# Autodesk Inventor assembly: 全体v1
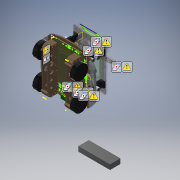
[picture p0: Inventor's stored thumbnail of the model, 180x180]
Saved by Autodesk Inventor 2018.3 (Build 223284000, 284)
## iProperties
Created: 2018-11-27
Part Number: 全体v1
Material: 一般
Document SubType Name: Assembly
Designer: shun2
Author: shun2
## Documents named in this file (27)
- C:\Users\shun2\OneDrive\おそらく最新版(2018.7.31)\全体v1.iam
- C:\Users\shun2\OneDrive\おそらく最新版(2018.7.31)\ギアボックス\ギアボックスv2.iam
- C:\Users\shun2\OneDrive\おそらく最新版(2018.7.31)\1枚目\一枚目.ipt
- C:\Users\shun2\OneDrive\おそらく最新版(2018.7.31)\基板保護2018.8.7.ipt
- C:\Users\shun2\OneDrive\おそらく最新版(2018.7.31)\2枚目\2枚目.ipt
- C:\Users\shun2\OneDrive\おそらく最新版(2018.7.31)\3枚目\3枚目v4.ipt
- C:\Users\shun2\OneDrive\おそらく最新版(2018.7.31)\ping-module.iam
- C:\Users\shun2\OneDrive\おそらく最新版(2018.7.31)\pingmodule-y.iam
- C:\Users\shun2\OneDrive\おそらく最新版(2018.7.31)\Color.ipt
- C:\Users\shun2\OneDrive\おそらく最新版(2018.7.31)\モタドラ.ipt
- C:\Users\shun2\OneDrive\おそらく最新版(2018.7.31)\メイン基板.ipt
- C:\Users\shun2\OneDrive\おそらく最新版(2018.7.31)\Aquila-2018-Under.ipt
- C:\Users\shun2\OneDrive\おそらく最新版(2018.7.31)\LiFePo.ipt
- C:\Users\shun2\OneDrive\おそらく最新版(2018.7.31)\LiFeGuard.ipt
- C:\Users\shun2\OneDrive\おそらく最新版(2018.7.31)\Ping-front.ipt
- C:\Users\shun2\OneDrive\おそらく最新版(2018.7.31)\Tire.ipt
- C:\Users\shun2\OneDrive\おそらく最新版(2018.7.31)\レスキューキット投下機構\RescueKit-Pipev3.ipt
- C:\Users\shun2\OneDrive\おそらく最新版(2018.7.31)\レスキューキット投下機構\RescueKit-Slidev2.ipt
- C:\Users\shun2\OneDrive\おそらく最新版(2018.7.31)\レスキューキット投下機構\28BYJ-48.ipt
- C:\Users\shun2\OneDrive\おそらく最新版(2018.7.31)\レスキューキット投下機構\RescueKit-Gear-18.ipt
- C:\Users\shun2\OneDrive\おそらく最新版(2018.7.31)\UI固定具.ipt
- C:\Users\shun2\OneDrive\おそらく最新版(2018.7.31)\M024-ILI9328 data.ipt
- C:\Users\shun2\OneDrive\おそらく最新版(2018.7.31)\GyroMountv2.ipt
- C:\Users\shun2\OneDrive\おそらく最新版(2018.7.31)\OpenMVMount-Tate-Shortv2.ipt
- C:\Users\shun2\OneDrive\おそらく最新版(2018.7.31)\OpenMVMount-Tatev2.ipt
- C:\Users\shun2\OneDrive\おそらく最新版(2018.7.31)\ping.ipt
- C:\Users\shun2\OneDrive\おそらく最新版(2018.7.31)\ガイド\ガイド横上.ipt
## Components (34 placed, 26 different names)
1. 一枚目:1 — メイト:1, メイト:2, フラッシュ:1, フラッシュ:2, フラッシュ:3, フラッシュ:4, メイト:3, メイト:4, メイト:5, メイト:44, メイト:45, メイト:46, メイト:47, メイト:48, メイト:49, メイト:53, メイト:54, メイト:55, メイト:95, メイト:151
2. 2枚目:1 — メイト:6, メイト:7, メイト:8, メイト:41, メイト:42, メイト:94, メイト:108, メイト:109, メイト:110, メイト:127, メイト:157, メイト:158, メイト:179, メイト:180, メイト:181, メイト:187, メイト:188, メイト:189, メイト:190, メイト:191, メイト:192
3. 3枚目v4:1 — メイト:41, メイト:42, メイト:50, メイト:94, メイト:127, メイト:132, メイト:133, メイト:134, メイト:135, メイト:136, メイト:137, メイト:138, メイト:139, メイト:140, メイト:141, メイト:142, メイト:143, メイト:144, メイト:145, メイト:146, メイト:159, メイト:160, メイト:161, メイト:162, メイト:163, メイト:164, メイト:165, メイト:166, メイト:177, メイト:178, メイト:182, メイト:183
4. 基板保護2018.8.7:1 — メイト:3, メイト:4, メイト:5, メイト:6, メイト:7, メイト:8
5. LiFePo:1
6. LiFeGuard:2 — メイト:108, メイト:109, メイト:110
7. RescueKit-Slidev2:1 — メイト:157
8. 28BYJ-48:1 — メイト:152, メイト:153, メイト:158
9. RescueKit-Gear-18:1 — メイト:152, メイト:153
10. RescueKit-Pipev3:1 — メイト:159, メイト:160, メイト:161
11. UI固定具:1 — メイト:164, メイト:165, メイト:166, メイト:168, メイト:169, メイト:170, メイト:171, メイト:172, メイト:173
12. M024-ILI9328 data:1 — メイト:168, メイト:169, メイト:170
13. GyroMountv2:1 — メイト:171, メイト:172, メイト:173
14. OpenMVMount-Tatev2:1 — メイト:177, メイト:178
15. Ping-front:1 — メイト:179, メイト:180, メイト:181, メイト:184, メイト:185, メイト:186
16. OpenMVMount-Tate-Shortv2:1 — メイト:182, メイト:183
17. ping:1 — メイト:184, メイト:185, メイト:186
18. ガイド横上:1 — メイト:187, メイト:188, メイト:189
19. ガイド横上:2 — メイト:190, メイト:191, メイト:192
20. ping-module:1 [sub-assembly] — メイト:132, メイト:133, メイト:134
21. ping-module:2 [sub-assembly] — メイト:141, メイト:142, メイト:143
22. ping-module:3 [sub-assembly] — メイト:138, メイト:139, メイト:140
23. ping-module:4 [sub-assembly] — メイト:135, メイト:136, メイト:137
24. pingmodule-y:1 [sub-assembly] — メイト:144, メイト:145, メイト:146
25. Color:1 — メイト:44, メイト:45, メイト:46
26. モタドラ:1 — メイト:47, メイト:48, メイト:49
27. メイン基板:1 — メイト:50, メイト:162, メイト:163
28. Aquila-2018-Under:2 — メイト:53, メイト:54, メイト:55
29. Tire:1 — メイト:86, メイト:87
30. Tire:2 — メイト:88, メイト:89
31. Tire:3 — メイト:92, メイト:93
32. Tire:4 — メイト:90, メイト:91
33. ギアボックスv2:2 [sub-assembly] — メイト:2, フラッシュ:1, フラッシュ:4, メイト:86, メイト:87, メイト:88, メイト:89
34. ギアボックスv2:1 [sub-assembly] — メイト:1, フラッシュ:2, フラッシュ:3, メイト:90, メイト:91, メイト:92, メイト:93, メイト:96
## Relationships (89: Mate 85, Flush 4)
- メイト:1 [Mate] (3 mm): 一枚目:1 ↔ ギアボックスv2:1
- メイト:2 [Mate] (3 mm): 一枚目:1 ↔ ギアボックスv2:2
- フラッシュ:1 [Flush]: 一枚目:1 ↔ ギアボックスv2:2
- フラッシュ:2 [Flush]: 一枚目:1 ↔ ギアボックスv2:1
- フラッシュ:3 [Flush] (2 mm): 一枚目:1 ↔ ギアボックスv2:1
- フラッシュ:4 [Flush] (2 mm): 一枚目:1 ↔ ギアボックスv2:2
- メイト:3 [Mate] (0.2 mm): 一枚目:1 ↔ 基板保護2018.8.7:1
- メイト:4 [Mate]: 一枚目:1 ↔ 基板保護2018.8.7:1
- メイト:5 [Mate]: 一枚目:1 ↔ 基板保護2018.8.7:1
- メイト:6 [Mate] (3 mm): 2枚目:1 ↔ 基板保護2018.8.7:1
- メイト:7 [Mate]: 2枚目:1 ↔ 基板保護2018.8.7:1
- メイト:8 [Mate]: 2枚目:1 ↔ 基板保護2018.8.7:1
- メイト:41 [Mate] (80 mm): 2枚目:1 ↔ 3枚目v4:1
- メイト:42 [Mate]: 2枚目:1 ↔ 3枚目v4:1
- メイト:44 [Mate] (40 mm): 一枚目:1 ↔ Color:1
- メイト:45 [Mate]: 一枚目:1 ↔ Color:1
- メイト:46 [Mate]: 一枚目:1 ↔ Color:1
- メイト:47 [Mate] (8 mm): 一枚目:1 ↔ モタドラ:1
- メイト:48 [Mate]: 一枚目:1 ↔ モタドラ:1
- メイト:49 [Mate]: 一枚目:1 ↔ モタドラ:1
- メイト:50 [Mate] (8 mm): 3枚目v4:1 ↔ メイン基板:1
- メイト:53 [Mate] (3 mm): 一枚目:1 ↔ Aquila-2018-Under:2
- メイト:54 [Mate]: 一枚目:1 ↔ Aquila-2018-Under:2
- メイト:55 [Mate]: 一枚目:1 ↔ Aquila-2018-Under:2
- メイト:86 [Mate] (8 mm): Tire:1 ↔ ギアボックスv2:2
- メイト:87 [Mate]: Tire:1 ↔ ギアボックスv2:2
- メイト:88 [Mate] (8 mm): Tire:2 ↔ ギアボックスv2:2
- メイト:89 [Mate]: Tire:2 ↔ ギアボックスv2:2
- メイト:90 [Mate]: Tire:4 ↔ ギアボックスv2:1
- メイト:91 [Mate] (8 mm): Tire:4 ↔ ギアボックスv2:1
- メイト:92 [Mate]: Tire:3 ↔ ギアボックスv2:1
- メイト:93 [Mate] (8 mm): Tire:3 ↔ ギアボックスv2:1
- メイト:94 [Mate]: 2枚目:1 ↔ 3枚目v4:1
- メイト:95 [Mate]: 一枚目:1
- メイト:96 [Mate]: ギアボックスv2:1
- メイト:108 [Mate]: 2枚目:1 ↔ LiFeGuard:2
- メイト:109 [Mate]: 2枚目:1 ↔ LiFeGuard:2
- メイト:110 [Mate]: 2枚目:1 ↔ LiFeGuard:2
- メイト:127 [Mate]: 2枚目:1 ↔ 3枚目v4:1
- メイト:132 [Mate]: 3枚目v4:1 ↔ ping-module:1
- メイト:133 [Mate]: 3枚目v4:1 ↔ ping-module:1
- メイト:134 [Mate]: 3枚目v4:1 ↔ ping-module:1
- メイト:135 [Mate]: 3枚目v4:1 ↔ ping-module:4
- メイト:136 [Mate]: 3枚目v4:1 ↔ ping-module:4
- メイト:137 [Mate]: 3枚目v4:1 ↔ ping-module:4
- メイト:138 [Mate]: 3枚目v4:1 ↔ ping-module:3
- メイト:139 [Mate]: 3枚目v4:1 ↔ ping-module:3
- メイト:140 [Mate]: 3枚目v4:1 ↔ ping-module:3
- メイト:141 [Mate]: 3枚目v4:1 ↔ ping-module:2
- メイト:142 [Mate]: 3枚目v4:1 ↔ ping-module:2
- メイト:143 [Mate]: 3枚目v4:1 ↔ ping-module:2
- メイト:144 [Mate]: 3枚目v4:1 ↔ pingmodule-y:1
- メイト:145 [Mate]: 3枚目v4:1 ↔ pingmodule-y:1
- メイト:146 [Mate]: 3枚目v4:1 ↔ pingmodule-y:1
- メイト:151 [Mate]: 一枚目:1
- メイト:152 [Mate]: 28BYJ-48:1 ↔ RescueKit-Gear-18:1
- メイト:153 [Mate] (5 mm): 28BYJ-48:1 ↔ RescueKit-Gear-18:1
- メイト:157 [Mate]: 2枚目:1 ↔ RescueKit-Slidev2:1
- メイト:158 [Mate] (11 mm): 2枚目:1 ↔ 28BYJ-48:1
- メイト:159 [Mate]: 3枚目v4:1 ↔ RescueKit-Pipev3:1
- メイト:160 [Mate]: 3枚目v4:1 ↔ RescueKit-Pipev3:1
- メイト:161 [Mate]: 3枚目v4:1 ↔ RescueKit-Pipev3:1
- メイト:162 [Mate]: 3枚目v4:1 ↔ メイン基板:1
- メイト:163 [Mate]: 3枚目v4:1 ↔ メイン基板:1
- メイト:164 [Mate]: 3枚目v4:1 ↔ UI固定具:1
- メイト:165 [Mate]: 3枚目v4:1 ↔ UI固定具:1
- メイト:166 [Mate]: 3枚目v4:1 ↔ UI固定具:1
- メイト:168 [Mate]: UI固定具:1 ↔ M024-ILI9328 data:1
- メイト:169 [Mate]: UI固定具:1 ↔ M024-ILI9328 data:1
- メイト:170 [Mate] (2 mm): UI固定具:1 ↔ M024-ILI9328 data:1
- メイト:171 [Mate] (25 mm): UI固定具:1 ↔ GyroMountv2:1
- メイト:172 [Mate]: UI固定具:1 ↔ GyroMountv2:1
- メイト:173 [Mate]: UI固定具:1 ↔ GyroMountv2:1
- メイト:177 [Mate]: 3枚目v4:1 ↔ OpenMVMount-Tatev2:1
- メイト:178 [Mate]: 3枚目v4:1 ↔ OpenMVMount-Tatev2:1
- メイト:179 [Mate]: 2枚目:1 ↔ Ping-front:1
- メイト:180 [Mate]: 2枚目:1 ↔ Ping-front:1
- メイト:181 [Mate]: 2枚目:1 ↔ Ping-front:1
- メイト:182 [Mate]: 3枚目v4:1 ↔ OpenMVMount-Tate-Shortv2:1
- メイト:183 [Mate]: 3枚目v4:1 ↔ OpenMVMount-Tate-Shortv2:1
- メイト:184 [Mate]: Ping-front:1 ↔ ping:1
- メイト:185 [Mate] (1 mm): Ping-front:1 ↔ ping:1
- メイト:186 [Mate]: Ping-front:1 ↔ ping:1
- メイト:187 [Mate] (-5.5 mm): 2枚目:1 ↔ ガイド横上:1
- メイト:188 [Mate]: 2枚目:1 ↔ ガイド横上:1
- メイト:189 [Mate]: 2枚目:1 ↔ ガイド横上:1
- メイト:190 [Mate]: 2枚目:1 ↔ ガイド横上:2
- メイト:191 [Mate]: 2枚目:1 ↔ ガイド横上:2
- メイト:192 [Mate]: 2枚目:1 ↔ ガイド横上:2
